# Autodesk Inventor assembly: Clutch02
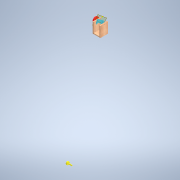
[picture p0: Inventor's stored thumbnail of the model, 180x180]
Saved by Autodesk Inventor 2021 (Build 250183000, 183)
## iProperties
Created: 2020-07-03
Part Number: Clutch02
Document SubType Name: Assembly
Designer: robst
Author: robst
## Documents named in this file (6)
- C:\git\CAD-Development\robSteele\ShapeWays\TelescopeProjects\TelescopeMount\Clutch02.iam
- C:\git\CAD-Development\robSteele\ShapeWays\TelescopeProjects\TelescopeMount\clutch02-forkBase.ipt
- C:\git\CAD-Development\robSteele\ShapeWays\TelescopeProjects\TelescopeMount\tubeBracketV02.ipt
- C:\git\CAD-Development\robSteele\ShapeWays\TelescopeProjects\TelescopeMount\clutch02-simplyGearDisk.ipt
- C:\git\CAD-Development\robSteele\ShapeWays\TelescopeProjects\TelescopeMount\clutch02-releaseMechanism.ipt
- C:\git\CAD-Development\robSteele\ShapeWays\TelescopeProjects\TelescopeMount\Compress Spring11.ipt
## Components (5 placed, 5 different names)
1. clutch02-forkBase:1 — Insert:1, Flush:1
2. tubeBracketV02:1 — Insert:1
3. clutch02-simplyGearDisk:1 — Flush:1, Flush:2, Flush:3, Flush:5
4. clutch02-releaseMechanism:1 — Flush:2, Flush:3, Mate:1, Flush:4, Flush:5
5. Compress Spring1:1 — Mate:1, Flush:4
## Relationships (7: Flush 5, Insert 1, Mate 1)
- Insert:1 (25.4 mm): clutch02-forkBase:1 ↔ tubeBracketV02:1
- Flush:1 (6.35 mm): clutch02-forkBase:1 ↔ clutch02-simplyGearDisk:1
- Flush:2: clutch02-simplyGearDisk:1 ↔ clutch02-releaseMechanism:1
- Flush:3: clutch02-simplyGearDisk:1 ↔ clutch02-releaseMechanism:1
- Mate:1: clutch02-releaseMechanism:1 ↔ Compress Spring1:1
- Flush:4: clutch02-releaseMechanism:1 ↔ Compress Spring1:1
- Flush:5: clutch02-simplyGearDisk:1 ↔ clutch02-releaseMechanism:1
